# Autodesk Inventor assembly: Robot
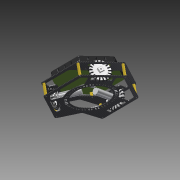
[picture p0: Inventor's stored thumbnail of the model, 180x180]
Saved by Autodesk Inventor 2015 (Build 190159000, 159)
## iProperties
Created: 2016-10-01
Part Number: Robot
Document SubType Name: Assembly
Designer: James Yelland
Author: James Yelland
## Documents named in this file (10)
- C:\Users\James Yelland\git\LJ-STAND\Design\Models\Version 2\Robot.iam
- C:\Users\James Yelland\git\LJ-STAND\Design\Models\Version 2\Bottom Plate.ipt
- C:\Users\James Yelland\git\LJ-STAND\Design\Models\Version 2\Middle Plate.ipt
- C:\Users\James Yelland\git\LJ-STAND\Design\Models\Common\Standoff 30.ipt
- C:\Users\James Yelland\git\LJ-STAND\Design\Models\Version 2\Motor Mount.ipt
- C:\Users\James Yelland\git\LJ-STAND\Design\Models\Common\Motor.ipt
- C:\Users\James Yelland\git\LJ-STAND\Design\Models\Common\Wheel.ipt
- C:\Users\James Yelland\git\LJ-STAND\Design\Models\Common\Standoff 10.ipt
- C:\Users\James Yelland\git\LJ-STAND\Design\Models\Version 2\PCB.ipt
- C:\Users\James Yelland\git\LJ-STAND\Design\Models\Version 2\TSOP Cover Ring.ipt
## Components (23 placed, 9 different names)
1. Bottom Plate:1 — Mate:1, Mate:2, Mate:3, Mate:4, Mate:5, Mate:6, Mate:7, Mate:8, Mate:12, Mate:13, Mate:14, Mate:15, Mate:16, Mate:17, Mate:18, Mate:19, Mate:20, Mate:53, Mate:54, Mate:55, Mate:56
2. Middle Plate:1 — Mate:9, Mate:10, Mate:11, Mate:61, Mate:62, Insert:1, Insert:2, Insert:3, Insert:4
3. Standoff 30:1 — Mate:4, Mate:5
4. Standoff 30:2 — Mate:3, Mate:6, Mate:9, Mate:11
5. Standoff 30:3 — Mate:2, Mate:8
6. Standoff 30:4 — Mate:1, Mate:7, Mate:10
7. Motor Mount:1 — Mate:12, Mate:13, Mate:14, Mate:22, Mate:24, Mate:28
8. Motor Mount:2 — Mate:15, Mate:16, Mate:17, Mate:21, Mate:25, Mate:29
9. Motor Mount:3 — Mate:18, Mate:19, Mate:20, Mate:23, Mate:26, Mate:27
10. Motor:1 — Mate:22, Mate:24, Mate:28, Mate:30, Flush:3
11. Motor:2 — Mate:23, Mate:26, Mate:27, Mate:31, Flush:2
12. Motor:3 — Mate:21, Mate:25, Mate:29, Mate:32, Flush:1
13. Wheel:1 — Mate:30, Flush:3
14. Wheel:2 — Mate:31, Flush:2
15. Wheel:3 — Mate:32, Flush:1
16. PCB:1 — Insert:5, Mate:63, Mate:64, Mate:65, Mate:66
17. Standoff 30:5 — Mate:53, Mate:56
18. Standoff 30:6 — Mate:54, Mate:55
19. Standoff 10:1 — Mate:61, Insert:4
20. Standoff 10:2 — Insert:2, Mate:63
21. Standoff 10:3 — Insert:1, Insert:5
22. Standoff 10:4 — Mate:62, Insert:3
23. TSOP Cover Ring:1 — Mate:64, Mate:65, Mate:66
## Relationships (50: Mate 42, Insert 5, Flush 3)
- Mate:1: Bottom Plate:1 ↔ Standoff 30:4
- Mate:2: Bottom Plate:1 ↔ Standoff 30:3
- Mate:3: Bottom Plate:1 ↔ Standoff 30:2
- Mate:4: Bottom Plate:1 ↔ Standoff 30:1
- Mate:5: Bottom Plate:1 ↔ Standoff 30:1
- Mate:6: Bottom Plate:1 ↔ Standoff 30:2
- Mate:7: Bottom Plate:1 ↔ Standoff 30:4
- Mate:8: Bottom Plate:1 ↔ Standoff 30:3
- Mate:9: Middle Plate:1 ↔ Standoff 30:2
- Mate:10: Middle Plate:1 ↔ Standoff 30:4
- Mate:11: Middle Plate:1 ↔ Standoff 30:2
- Mate:12: Bottom Plate:1 ↔ Motor Mount:1
- Mate:13: Bottom Plate:1 ↔ Motor Mount:1
- Mate:14: Bottom Plate:1 ↔ Motor Mount:1
- Mate:15: Bottom Plate:1 ↔ Motor Mount:2
- Mate:16: Bottom Plate:1 ↔ Motor Mount:2
- Mate:17: Bottom Plate:1 ↔ Motor Mount:2
- Mate:18: Bottom Plate:1 ↔ Motor Mount:3
- Mate:19: Bottom Plate:1 ↔ Motor Mount:3
- Mate:20: Bottom Plate:1 ↔ Motor Mount:3
- Mate:21: Motor Mount:2 ↔ Motor:3
- Mate:22: Motor Mount:1 ↔ Motor:1
- Mate:23: Motor Mount:3 ↔ Motor:2
- Mate:24: Motor Mount:1 ↔ Motor:1
- Mate:25: Motor Mount:2 ↔ Motor:3
- Mate:26: Motor Mount:3 ↔ Motor:2
- Mate:27: Motor Mount:3 ↔ Motor:2
- Mate:28: Motor Mount:1 ↔ Motor:1
- Mate:29: Motor Mount:2 ↔ Motor:3
- Mate:30: Motor:1 ↔ Wheel:1
- Mate:31: Motor:2 ↔ Wheel:2
- Mate:32: Motor:3 ↔ Wheel:3
- Flush:1 (-7 mm): Motor:3 ↔ Wheel:3
- Flush:2 (-7 mm): Motor:2 ↔ Wheel:2
- Flush:3 (-7 mm): Motor:1 ↔ Wheel:1
- Mate:53: Bottom Plate:1 ↔ Standoff 30:5
- Mate:54: Bottom Plate:1 ↔ Standoff 30:6
- Mate:55: Bottom Plate:1 ↔ Standoff 30:6
- Mate:56: Bottom Plate:1 ↔ Standoff 30:5
- Mate:61: Middle Plate:1 ↔ Standoff 10:1
- Mate:62: Middle Plate:1 ↔ Standoff 10:4
- Insert:1: Middle Plate:1 ↔ Standoff 10:3
- Insert:2: Middle Plate:1 ↔ Standoff 10:2
- Insert:3: Middle Plate:1 ↔ Standoff 10:4
- Insert:4: Middle Plate:1 ↔ Standoff 10:1
- Insert:5: PCB:1 ↔ Standoff 10:3
- Mate:63: PCB:1 ↔ Standoff 10:2
- Mate:64: PCB:1 ↔ TSOP Cover Ring:1
- Mate:65: PCB:1 ↔ TSOP Cover Ring:1
- Mate:66: PCB:1 ↔ TSOP Cover Ring:1
